# Autodesk Inventor assembly: Filter Housing Exhaust
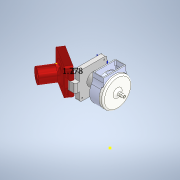
[picture p0: Inventor's stored thumbnail of the model, 180x180]
Saved by Autodesk Inventor 2020 (Build 240168000, 168)
## iProperties
Created: 2020-04-09
Part Number: Filter Housing Exhaust
Document SubType Name: Assembly
Designer: Simon
Author: Simon
## Documents named in this file (4)
- \\Mac\Home\Desktop\3D\Breeze thing\Filter housing with o ring\assembled exhaust filter housing.iam
- \\Mac\Home\Desktop\3D\Breeze thing\Filter housing with o ring\exhaustFilterHousing.iam
- \\Mac\Home\Desktop\3D\Breeze thing\Filter housing with o ring\clip.ipt
- \\Mac\Home\Desktop\3D\Breeze thing\Filter housing with o ring\filter_connector v1 (1).ipt
## Components (3 placed, 3 different names)
1. exhaustFilterHousing:1 [sub-assembly] — Mate:1, Mate:2, Mate:3, Mate:4, Mate:5
2. clip:1 — Mate:1, Mate:2, Mate:3
3. filter_connector v1 (1):1 — Mate:4, Mate:5
## Relationships (5: Mate 5)
- Mate:1: exhaustFilterHousing:1 ↔ clip:1
- Mate:2: exhaustFilterHousing:1 ↔ clip:1
- Mate:3: exhaustFilterHousing:1 ↔ clip:1
- Mate:4: exhaustFilterHousing:1 ↔ filter_connector v1 (1):1
- Mate:5 (0.25 mm): exhaustFilterHousing:1 ↔ filter_connector v1 (1):1
